# Autodesk Inventor assembly: Pistoni pinza - Trasporto
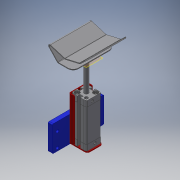
[picture p0: Inventor's stored thumbnail of the model, 180x180]
Saved by Autodesk Inventor 2018 (Build 220112000, 112)
## iProperties
Created: 2020-05-30
Part Number: Pistoni pinza - Trasporto
Material: Generico
Document SubType Name: Weldment
Designer: Francesco
Weld Material: Welded Aluminum-6061
Author: Francesco
## Documents named in this file (6)
- C:\Users\Francesco\no-brim\Meccanica\Progetto Inventor no-brim\Assiemi\Pistoni pinza - Trasporto.iam
- C:\Users\Francesco\no-brim\Meccanica\Progetto Inventor no-brim\Parti\ADN 16 - 50 A-P-A #536331\AIS2017\536331 ADN-16-50-A-P-A---(asm_0).iam
- C:\Users\Francesco\no-brim\Meccanica\Progetto Inventor no-brim\Parti\Supporto pistone pinza.ipt
- C:\Users\Francesco\no-brim\Meccanica\Progetto Inventor no-brim\Unificati\it-IT\ISO 4035(2)\ISO 4035 - M8 - ISO.ipt
- C:\Users\Francesco\no-brim\Meccanica\Progetto Inventor no-brim\Parti\Lamiera pinza.ipt
- C:\Users\Francesco\no-brim\Meccanica\Progetto Inventor no-brim\Parti\Piastra collegamento asse - pistone.ipt
## Components (6 placed, 5 different names)
1. 536331 ADN-16-50-A-P-A---(asm_0):1 [sub-assembly] — Coincidente:1, Coincidente:2, Coincidente:3, Coincidente:5, Allineato:1, Coincidente:8, Coincidente:9, Angolo:1
2. Supporto pistone pinza:1 — Coincidente:1, Coincidente:2, Coincidente:3, Coincidente:12, Allineato:2, Coincidente:13
3. ISO 4035 M8:1 — Coincidente:5, Coincidente:6, Coincidente:10
4. ISO 4035 M8:2 — Coincidente:8, Coincidente:11
5. Lamiera pinza:1 — Coincidente:9, Coincidente:10, Coincidente:11, Angolo:1
6. Piastra collegamento asse - pistone:1 — Coincidente:12, Allineato:2, Coincidente:13
## Relationships (14: Mate 11, Flush 2, Angle 1)
- Coincidente:1 [Mate]: 536331 ADN-16-50-A-P-A---(asm_0):1 ↔ Supporto pistone pinza:1
- Coincidente:2 [Mate]: 536331 ADN-16-50-A-P-A---(asm_0):1 ↔ Supporto pistone pinza:1
- Coincidente:3 [Mate]: 536331 ADN-16-50-A-P-A---(asm_0):1 ↔ Supporto pistone pinza:1
- Coincidente:5 [Mate]: 536331 ADN-16-50-A-P-A---(asm_0):1 ↔ ISO 4035 M8:1
- Allineato:1 [Flush] (-9 mm): 536331 ADN-16-50-A-P-A---(asm_0):1
- Coincidente:6 [Mate]: ISO 4035 M8:1
- Coincidente:8 [Mate]: 536331 ADN-16-50-A-P-A---(asm_0):1 ↔ ISO 4035 M8:2
- Coincidente:9 [Mate]: 536331 ADN-16-50-A-P-A---(asm_0):1 ↔ Lamiera pinza:1
- Coincidente:10 [Mate]: ISO 4035 M8:1 ↔ Lamiera pinza:1
- Coincidente:11 [Mate]: ISO 4035 M8:2 ↔ Lamiera pinza:1
- Angolo:1 [Angle] (0 deg): 536331 ADN-16-50-A-P-A---(asm_0):1 ↔ Lamiera pinza:1
- Coincidente:12 [Mate]: Supporto pistone pinza:1 ↔ Piastra collegamento asse - pistone:1
- Allineato:2 [Flush]: Supporto pistone pinza:1 ↔ Piastra collegamento asse - pistone:1
- Coincidente:13 [Mate]: Supporto pistone pinza:1 ↔ Piastra collegamento asse - pistone:1
